# Autodesk Inventor assembly: ASY МОО 001 отстойник осветлитель
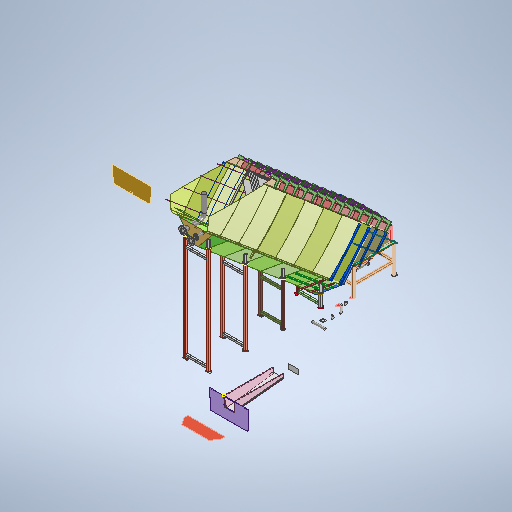
[picture p0: Inventor's stored thumbnail of the model, 512x512]
Saved by Autodesk Inventor 2025 (Build 290162010, 162A)
## iProperties
Created: 2024-04-28
Part Number: ASY МОО 001 отстойник осветлитель
Document SubType Name: Weldment
Designer: admin
Weld Material: Welded Aluminum-6061
Mass: 3.05393e+07 g
Surface Area: 3.06781e+06 cm^2
Volume: 2.84022e+07 cm^3
Density: 1.07525 g/cm^3
Author: admin
## Documents named in this file (70)
- C:\Users\pokla\Documents\Inventor\Отстойник осветлитель\Manturovo_Se-clar-Gleb\ASY MSC 001 отстойник осветлитель.iam
- C:\Users\pokla\Documents\Inventor\Отстойник осветлитель\Manturovo_Se-clar-Gleb\Рама основания\ASY MSC 090 base frame.iam
- C:\Users\pokla\Documents\Inventor\Отстойник осветлитель\Manturovo_Se-clar-Gleb\ASY MSC 080 roсket.iam
- C:\Users\pokla\Documents\Inventor\Отстойник осветлитель\Manturovo_Se-clar-Gleb\ASY MSC 010 cone.iam
- C:\Users\pokla\Documents\Inventor\Отстойник осветлитель\Manturovo_Se-clar-Gleb\ракета\МОО 064 ракета труба.ipt
- C:\Users\pokla\Documents\Inventor\Отстойник осветлитель\Manturovo_Se-clar-Gleb\MSC 000 DIM settler-clarifier.ipt
- C:\Users\pokla\Documents\Inventor\Отстойник осветлитель\Manturovo_Se-clar-Gleb\MSC 031 sheet lowerback.ipt
- C:\Users\pokla\Documents\Inventor\Отстойник осветлитель\Manturovo_Se-clar-Gleb\MSC 021 sheet left board hip.ipt
- C:\Users\pokla\Documents\Inventor\Отстойник осветлитель\Manturovo_Se-clar-Gleb\MSC 022 sheet right board hip.ipt
- C:\Users\pokla\Documents\Inventor\Отстойник осветлитель\Manturovo_Se-clar-Gleb\конус\MSC 071 ridge 1.ipt
- C:\Users\pokla\Documents\Inventor\Отстойник осветлитель\Manturovo_Se-clar-Gleb\конус\MSC 073 ridge 3.ipt
- C:\Users\pokla\Documents\Inventor\Отстойник осветлитель\Manturovo_Se-clar-Gleb\конус\MSC 074 face 1.ipt
- C:\Users\pokla\Documents\Inventor\Отстойник осветлитель\Manturovo_Se-clar-Gleb\Content Center Files\en-US\ISO 5251 B 3D\ISO 5251 Bends 3D without straight ends(90 deg) DN150 11 11.ipt
- C:\Users\pokla\Documents\Inventor\Отстойник осветлитель\Manturovo_Se-clar-Gleb\Content Center Files\en-US\DIN EN 1092-1 01 - PN 25\DIN EN 1092-1 Plate Flange for Welding Type 01 - PN 25 150 x 168.3.ipt
- C:\Users\pokla\Documents\Inventor\Отстойник осветлитель\Manturovo_Se-clar-Gleb\МОО 061 труба верх 1.ipt
- C:\Users\pokla\Documents\Inventor\Отстойник осветлитель\Manturovo_Se-clar-Gleb\МОО 062 труба верх 2.ipt
- C:\Users\pokla\Documents\Inventor\Отстойник осветлитель\Manturovo_Se-clar-Gleb\МОО 063 труба верх 3.ipt
- C:\Users\pokla\Documents\Inventor\Отстойник осветлитель\Manturovo_Se-clar-Gleb\Part1.ipt
- C:\Users\pokla\Documents\Inventor\Отстойник осветлитель\Manturovo_Se-clar-Gleb\MSC 0101 sheet gills.ipt
- C:\Users\pokla\Documents\Inventor\Отстойник осветлитель\Manturovo_Se-clar-Gleb\MSC 068 stringer lowerback.ipt
- C:\Users\pokla\Documents\Inventor\Отстойник осветлитель\Manturovo_Se-clar-Gleb\конус\MSC 072 ridge 2.ipt
- C:\Users\pokla\Documents\Inventor\Отстойник осветлитель\Manturovo_Se-clar-Gleb\MSC 075 face 2.ipt
- C:\Users\pokla\Documents\Inventor\Отстойник осветлитель\Manturovo_Se-clar-Gleb\MSC 076 face 3.ipt
- C:\Users\pokla\Documents\Inventor\Отстойник осветлитель\Manturovo_Se-clar-Gleb\MSC 077 face 4.ipt
- C:\Users\pokla\Documents\Inventor\Отстойник осветлитель\Manturovo_Se-clar-Gleb\MSC 110 revision hatch 1.ipt
- C:\Users\pokla\Documents\Inventor\Отстойник осветлитель\Manturovo_Se-clar-Gleb\MSC 035 ring.ipt
- C:\Users\pokla\Documents\Inventor\Отстойник осветлитель\Manturovo_Se-clar-Gleb\MSC 074 ridge 4.ipt
- C:\Users\pokla\Documents\Inventor\Отстойник осветлитель\Manturovo_Se-clar-Gleb\MSC 075 ridge 5.ipt
- C:\Users\pokla\Documents\Inventor\Отстойник осветлитель\Manturovo_Se-clar-Gleb\MSC 081 pillar 1.ipt
- C:\Users\pokla\Documents\Inventor\Отстойник осветлитель\Manturovo_Se-clar-Gleb\MSC 036 flange 500.ipt
- C:\Users\pokla\Documents\Inventor\Отстойник осветлитель\Manturovo_Se-clar-Gleb\MSC 037 flange cover 500.ipt
- C:\Users\pokla\Documents\Inventor\Отстойник осветлитель\Manturovo_Se-clar-Gleb\MSC 038 flange cover ring 500.ipt
- C:\Users\pokla\Documents\Inventor\Отстойник осветлитель\Manturovo_Se-clar-Gleb\MSC 039 flange cover plate 500.ipt
- C:\Users\pokla\Documents\Inventor\Отстойник осветлитель\Manturovo_Se-clar-Gleb\Рама основания\ASY MSC 120  base frame.iam
- C:\Users\pokla\Documents\Inventor\Отстойник осветлитель\Manturovo_Se-clar-Gleb\Рама основания\ASY MSC 121  base frame.iam
- C:\Users\pokla\Documents\Inventor\Отстойник осветлитель\Manturovo_Se-clar-Gleb\Чертеж для парам. рамы.ipt
- C:\Users\pokla\Documents\Inventor\Отстойник осветлитель\Manturovo_Se-clar-Gleb\ASY MSC 120.1  base frame.iam
- C:\Users\pokla\Documents\Inventor\Отстойник осветлитель\Manturovo_Se-clar-Gleb\ASY MSC 122  base frame.iam
- C:\Users\pokla\Documents\Inventor\Отстойник осветлитель\Manturovo_Se-clar-Gleb\ASY MSC 201 BACK.iam
- C:\Users\pokla\Documents\Inventor\Отстойник осветлитель\Manturovo_Se-clar-Gleb\ASY MSC 202 LEFT BOARD.iam
- C:\Users\pokla\Documents\Inventor\Отстойник осветлитель\Manturovo_Se-clar-Gleb\ASY MSC 203 RIGHT BOARD.iam
- C:\Users\pokla\Documents\Inventor\Отстойник осветлитель\Manturovo_Se-clar-Gleb\ASY MSC 204 BELLY.iam
- C:\Users\pokla\Documents\Inventor\Отстойник осветлитель\Manturovo_Se-clar-Gleb\MSC 063 stringer board #.ipt
- C:\Users\pokla\Documents\Inventor\Отстойник осветлитель\Manturovo_Se-clar-Gleb\MSC 064 stringer board ##.ipt
- C:\Users\pokla\Documents\Inventor\Отстойник осветлитель\Manturovo_Se-clar-Gleb\MSC 055 rib hip 2.ipt
- C:\Users\pokla\Documents\Inventor\Отстойник осветлитель\Manturovo_Se-clar-Gleb\MSC 054 rib hip 1.ipt
- C:\Users\pokla\Documents\Inventor\Отстойник осветлитель\Manturovo_Se-clar-Gleb\MSC 0102 sheet gills.ipt
- C:\Users\pokla\Documents\Inventor\Отстойник осветлитель\Manturovo_Se-clar-Gleb\MSC 078 creen pillar.iam
- C:\Users\pokla\Documents\Inventor\Отстойник осветлитель\Manturovo_Se-clar-Gleb\MSC 0202 sheet gills.ipt
- C:\Users\pokla\Documents\Inventor\Отстойник осветлитель\Manturovo_Se-clar-Gleb\MSC 0103 sheet gills.ipt
- C:\Users\pokla\Documents\Inventor\Отстойник осветлитель\Manturovo_Se-clar-Gleb\MSC 0203 sheet gills.ipt
- C:\Users\pokla\Documents\Inventor\Отстойник осветлитель\Manturovo_Se-clar-Gleb\MSC 0104 sheet gills.ipt
- C:\Users\pokla\Documents\Inventor\Отстойник осветлитель\Manturovo_Se-clar-Gleb\MSC 0204 sheet gills.ipt
- C:\Users\pokla\Documents\Inventor\Отстойник осветлитель\Manturovo_Se-clar-Gleb\MSC 0105 sheet gills.ipt
- C:\Users\pokla\Documents\Inventor\Отстойник осветлитель\Manturovo_Se-clar-Gleb\MSC 0205 sheet gills.ipt
- C:\Users\pokla\Documents\Inventor\Отстойник осветлитель\Manturovo_Se-clar-Gleb\MSC 0106 sheet gills.ipt
- C:\Users\pokla\Documents\Inventor\Отстойник осветлитель\Manturovo_Se-clar-Gleb\MSC 0206 sheet gills.ipt
- C:\Users\pokla\Documents\Inventor\Отстойник осветлитель\Manturovo_Se-clar-Gleb\MSC 0107 sheet gills.ipt
- C:\Users\pokla\Documents\Inventor\Отстойник осветлитель\Manturovo_Se-clar-Gleb\MSC 0207 sheet gills.ipt
- C:\Users\pokla\Documents\Inventor\Отстойник осветлитель\Manturovo_Se-clar-Gleb\MSC 079 creen pillar.ipt
- C:\Users\pokla\Documents\Inventor\Отстойник осветлитель\Manturovo_Se-clar-Gleb\ASY MSC 120 support.iam
- C:\Users\pokla\Documents\Inventor\Отстойник осветлитель\Manturovo_Se-clar-Gleb\ракета\МОО 065 ракета труба 5.ipt
- C:\Users\pokla\Documents\Inventor\Отстойник осветлитель\Manturovo_Se-clar-Gleb\ракета\МОО 066 ракета труба 6.ipt
- C:\Users\pokla\Documents\Inventor\Отстойник осветлитель\Manturovo_Se-clar-Gleb\ракета\МОО 067 ракета труба 7.ipt
- C:\Users\pokla\Documents\Inventor\Отстойник осветлитель\Manturovo_Se-clar-Gleb\ракета\МОО 068 ракета труба 8.ipt
- C:\Users\pokla\Documents\Inventor\Отстойник осветлитель\Manturovo_Se-clar-Gleb\ракета\МОО 069 ракета труба 9.ipt
- C:\Users\pokla\Documents\Inventor\Отстойник осветлитель\Manturovo_Se-clar-Gleb\Content Center Files\en-US\DIN EN 1092-1 01 - PN 25\DIN EN 1092-1 Plate Flange for Welding Type 01 - PN 25 80 x 88.9.ipt
- C:\Users\pokla\Documents\Inventor\Отстойник осветлитель\Manturovo_Se-clar-Gleb\MSC 0391 flange.ipt
- C:\Users\pokla\Documents\Inventor\Отстойник осветлитель\Manturovo_Se-clar-Gleb\MSC 0392 flange 2.ipt
- C:\Users\pokla\Documents\Inventor\Отстойник осветлитель\Manturovo_Se-clar-Gleb\ASY MSC 0130 cone exit back.iam
## Components (95 placed, 72 different names)
1. MSC 000 DIM settler-clarifier.ipt:1
2. MSC 001 DIM frame.ipt:1 — Flush:94, Mate:95, Mate:97, Mate:99, Mate:100
3. ASY MSC 120 support:1 [sub-assembly] — Mate:125, Cylindrical:6
4. ASY MSC 120 support:2 [sub-assembly] — Mate:129, Cylindrical:7
5. ASY MSC 120 support:3 [sub-assembly] — Mate:130, Cylindrical:8
6. ASY MSC 120 support:4 [sub-assembly] — Mate:131, Cylindrical:9
7. MSC 078 creen pillar:1 [sub-assembly]
8. ASY MSC 204 BELLY:1 [sub-assembly] — Mate:125, Mate:129, Mate:130, Mate:131, Mate:132, Mate:133, Mate:135, Flush:102, Mate:137, Mate:139
9. ASY MSC 203 RIGHT BOARD:1 [sub-assembly] — Mate:137, Mate:138
10. ASY MSC 202 LEFT BOARD:1 [sub-assembly]
11. ASY MSC 201 BACK:1 [sub-assembly] — Mate:134, Mate:138, Mate:139
12. ASY MSC 122  base frame:2 [sub-assembly] — Flush:97, Mate:102, Cylindrical:9
13. ASY MSC 120.1  base frame:2 [sub-assembly] — Flush:96, Mate:100, Mate:101, Cylindrical:7
14. ASY MSC 121  base frame:1 [sub-assembly] — Mate:98, Flush:95, Mate:99, Cylindrical:8
15. ASY MSC 120  base frame:1 [sub-assembly] — Flush:93, Mate:97, Cylindrical:6, Cylindrical:10
16. ASY MSC 080 roсket.iam:1 [sub-assembly] — Flush:23
17. ASY MSC 010 cone.iam:1 [sub-assembly] — Flush:22, Mate:16, Flush:28, Mate:65, Mate:78, Tangent:11, Flush:79, Mate:83, Flush:100
18. ASY MSC 090 base frame.iam:1 [sub-assembly] — Flush:19, Flush:21, Flush:82, Flush:100
19. МОО 064 ракета труба.ipt:1 — Rigid:212
20. MSC 031 sheet lowerback.ipt:1 — Mate:15, Mate:16, Tangent:10, Tangent:11, Tangent:12, Cylindrical:2, Rigid:185, Mate:134
21. MSC 021 sheet left board hip.ipt:1 — Flush:41, Mate:78
22. MSC 022 sheet right board hip.ipt:1 — Mate:30
23. MSC 071 ridge 1.ipt:1 — Mate:50, Rigid:211
24. MSC 073 ridge 3.ipt:1 — Rotational:6, Rigid:210, Rigid:211
25. MSC 072 ridge 2.ipt:1 — Rotational:6
26. MSC 077 face 4.ipt:1
27. MSC 074 ridge 4:1 — Rigid:210
28. MSC 075 ridge 5:1
29. MSC 074 face 1.ipt:1 — Rigid:156, Rigid:157, Flush:62, Rigid:159, Mate:132, Mate:133
30. МОО 061 труба верх 1.ipt:1 — Rigid:59, Rigid:159, Rotational:7
31. ISO 5251 Bends 3D without straight ends(90 deg) DN150 11 11.ipt:1 — Rigid:59, Rotational:2
32. МОО 062 труба верх 2.ipt:1 — Rigid:132, Rigid:156
33. DIN EN 1092-1 Plate Flange for Welding Type 01 - PN 25 150 x 168.3.ipt:2 — Rigid:132
34. МОО 063 труба верх 3.ipt:1 — Rigid:157, Rotational:5
35. Part1.ipt:1
36. MSC 068 stringer lowerback.ipt:1 — Mate:65, Tangent:10
37. МОО 061 труба верх 1.ipt:2 — Rotational:2
38. MSC 075 face 2.ipt:1 — Flush:61
39. MSC 076 face 3.ipt:1 — Flush:76
40. MSC 110 revision hatch 1:1 — Flush:82
41. MSC 068 stringer lowerback:2 — Mate:83, Tangent:12
42. MSC 035 ring:1 — Cylindrical:2, Rigid:185, Rigid:186
43. MSC 081 pillar 1:1
44. MSC 036 flange 500:1 — Rigid:175
45. MSC 036 flange 500:2 — Rigid:175, Rigid:176, Rigid:186
46. MSC 036 flange 500:3 — Rigid:176, Rigid:177, Mate:87
47. MSC 036 flange 500:4 — Rigid:177, Rotational:4
48. MSC 037 flange cover 500:1 — Rotational:4, Mate:87, Rigid:178, Mate:108
49. MSC 038 flange cover ring 500:1 — Rigid:178, Mate:109, Tangent:15
50. MSC 055 rib hip 2:2
51. MSC 063 stringer board #.ipt:2
52. MSC 064 stringer board ##.ipt:2
53. MSC 054 rib board hip 1:2
54. MSC 063 stringer board #.ipt:1
55. MSC 054 rib board hip 1:1
56. MSC 055 rib hip 2:1
57. MSC 064 stringer board ##.ipt:1
58. MSC 0102 sheet gills:1 — Rigid:197, Mate:124
59. MSC 0101 sheet gills.ipt:1
60. MSC 0202 sheet gills:1 — Rigid:197
61. MSC 0103 sheet gills:1 — Rigid:199, Mate:123, Mate:124
62. MSC 0203 sheet gills:1 — Rigid:199
63. MSC 0104 sheet gills:1 — Rigid:201, Mate:122, Mate:123
64. MSC 0204 sheet gills:1 — Rigid:201
65. MSC 0105 sheet gills:1 — Rigid:203, Mate:121, Mate:122
66. MSC 0205 sheet gills:1 — Rigid:203
67. MSC 0106 sheet gills:1 — Rigid:205, Mate:120, Mate:121
68. MSC 0206 sheet gills:1 — Rigid:205
69. MSC 0107 sheet gills:1 — Rigid:206, Mate:120
70. MSC 0207 sheet gills:1 — Rigid:206
71. MSC 079 creen pillar:2
72. МОО 064 ракета труба:2
73. МОО 065 ракета труба 5:1 — Rigid:209, Rotational:8
74. МОО 066 ракета труба 6:1
75. МОО 067 ракета труба 7:1 — Rigid:209
76. МОО 068 ракета труба 8:1
77. МОО 069 ракета труба 9:1
78. ASY MSC 120 support:5 [sub-assembly] — Cylindrical:10, Mate:135
79. DIN EN 1092-1 Plate Flange for Welding Type 01 - PN 25 80 x 88.9:1 — Rotational:5
80. DIN EN 1092-1 Plate Flange for Welding Type 01 - PN 25 150 x 168.3:3 — Rotational:7
81. MSC 0391 flange:1 — Rotational:8
82. MSC 0392 flange 2:1 — Rigid:212
83. ASY MSC 0130 cone exit back:1 [sub-assembly]
84. MSC 039 flange cover plate 500:1 — Mate:108, Mate:109, Tangent:15
85. MSC 039 flange cover plate 500:2
86. MSC 039 flange cover plate 500:3
87. MSC 039 flange cover plate 500:4
88. MSC 039 flange cover plate 500:5
89. MSC 039 flange cover plate 500:6
90. MSC 039 flange cover plate 500:7
91. MSC 039 flange cover plate 500:8
92. MSC 039 flange cover plate 500:9
93. MSC 039 flange cover plate 500:10
94. MSC 039 flange cover plate 500:11
95. MSC 039 flange cover plate 500:12
## Component patterns: (12 elements, first: MSC 039 flange cover plate 500:1)
## Relationships (102: Mate 38, WeldJoint 27, Flush 20, RevoluteJoint 6, CylindricalJoint 6, Tangent 4, Angle 1)
- [Flush]: ASY MSC 201 BACK:1
- Flush:19: ASY MSC 090 base frame.iam:1
- Flush:21: ASY MSC 090 base frame.iam:1
- Flush:22: ASY MSC 010 cone.iam:1
- Flush:23: ASY MSC 080 roсket.iam:1
- Mate:15: MSC 031 sheet lowerback.ipt:1
- Mate:16: ASY MSC 010 cone.iam:1 ↔ MSC 031 sheet lowerback.ipt:1
- Flush:28: ASY MSC 010 cone.iam:1
- [Flush]: ASY MSC 202 LEFT BOARD:1
- Flush:41: MSC 021 sheet left board hip.ipt:1
- Mate:30: MSC 022 sheet right board hip.ipt:1
- Mate:50 (200 mm): MSC 071 ridge 1.ipt:1
- Rigid:59 [WeldJoint]: МОО 061 труба верх 1.ipt:1 ↔ ISO 5251 Bends 3D without straight ends(90 deg) DN150 11 11.ipt:1
- Rigid:132 [WeldJoint]: МОО 062 труба верх 2.ipt:1 ↔ DIN EN 1092-1 Plate Flange for Welding Type 01 - PN 25 150 x 168.3.ipt:2
- Mate:65: ASY MSC 010 cone.iam:1 ↔ MSC 068 stringer lowerback.ipt:1
- [Mate]: ASY MSC 201 BACK:1 ↔ MSC 068 stringer lowerback.ipt:1
- Tangent:10: MSC 031 sheet lowerback.ipt:1 ↔ MSC 068 stringer lowerback.ipt:1
- Rotational:2 [RevoluteJoint]: ISO 5251 Bends 3D without straight ends(90 deg) DN150 11 11.ipt:1 ↔ МОО 061 труба верх 1.ipt:2
- Flush:61: MSC 075 face 2.ipt:1
- Rigid:156 [WeldJoint]: MSC 074 face 1.ipt:1 ↔ МОО 062 труба верх 2.ipt:1
- Rigid:157 [WeldJoint]: MSC 074 face 1.ipt:1 ↔ МОО 063 труба верх 3.ipt:1
- Flush:62: MSC 074 face 1.ipt:1
- Rigid:159 [WeldJoint] (-200 mm): MSC 074 face 1.ipt:1 ↔ МОО 061 труба верх 1.ipt:1
- Flush:76: MSC 076 face 3.ipt:1
- Mate:78: ASY MSC 010 cone.iam:1 ↔ MSC 021 sheet left board hip.ipt:1
- Tangent:11 (22 mm): ASY MSC 010 cone.iam:1 ↔ MSC 031 sheet lowerback.ipt:1
- Flush:79: ASY MSC 010 cone.iam:1
- Flush:82: ASY MSC 090 base frame.iam:1 ↔ MSC 110 revision hatch 1:1
- Mate:83: ASY MSC 010 cone.iam:1 ↔ MSC 068 stringer lowerback:2
- [Mate]: ASY MSC 201 BACK:1 ↔ MSC 068 stringer lowerback:2
- Tangent:12: MSC 031 sheet lowerback.ipt:1 ↔ MSC 068 stringer lowerback:2
- Rigid:175 [WeldJoint]: MSC 036 flange 500:1 ↔ MSC 036 flange 500:2
- Rigid:176 [WeldJoint]: MSC 036 flange 500:2 ↔ MSC 036 flange 500:3
- Rigid:177 [WeldJoint]: MSC 036 flange 500:3 ↔ MSC 036 flange 500:4
- Cylindrical:2: MSC 031 sheet lowerback.ipt:1 ↔ MSC 035 ring:1
- Rotational:4 [RevoluteJoint]: MSC 036 flange 500:4 ↔ MSC 037 flange cover 500:1
- Mate:87: MSC 036 flange 500:3 ↔ MSC 037 flange cover 500:1
- Rigid:178 [WeldJoint]: MSC 037 flange cover 500:1 ↔ MSC 038 flange cover ring 500:1
- Flush:93 (-3 mm): ASY MSC 120  base frame:1
- [Mate]: ASY MSC 120  base frame:1
- Flush:94: MSC 001 DIM frame.ipt:1
- Mate:95: MSC 001 DIM frame.ipt:1
- Mate:97: MSC 001 DIM frame.ipt:1 ↔ ASY MSC 120  base frame:1
- Mate:98: ASY MSC 121  base frame:1
- Flush:95 (-3 mm): ASY MSC 121  base frame:1
- Mate:99: MSC 001 DIM frame.ipt:1 ↔ ASY MSC 121  base frame:1
- Flush:96 (-3 mm): ASY MSC 120.1  base frame:2
- Mate:100: MSC 001 DIM frame.ipt:1 ↔ ASY MSC 120.1  base frame:2
- Mate:101: ASY MSC 120.1  base frame:2
- Flush:97 (-3 mm): ASY MSC 122  base frame:2
- Mate:102: ASY MSC 122  base frame:2
- Rigid:185 [WeldJoint] (20 mm): MSC 031 sheet lowerback.ipt:1 ↔ MSC 035 ring:1
- Mate:108: MSC 037 flange cover 500:1 ↔ MSC 039 flange cover plate 500:1
- Mate:109: MSC 038 flange cover ring 500:1 ↔ MSC 039 flange cover plate 500:1
- Tangent:15: MSC 038 flange cover ring 500:1 ↔ MSC 039 flange cover plate 500:1
- Rigid:186 [WeldJoint]: MSC 035 ring:1 ↔ MSC 036 flange 500:2
- [WeldJoint] (500 mm): MSC 054 rib board hip 1:1 ↔ MSC 055 rib hip 2:1
- [WeldJoint] (2 mm): ASY MSC 202 LEFT BOARD:1 ↔ MSC 064 stringer board ##.ipt:2
- [WeldJoint] (500 mm): ASY MSC 202 LEFT BOARD:1 ↔ MSC 055 rib hip 2:2
- [WeldJoint] (500 mm): MSC 055 rib hip 2:2 ↔ MSC 054 rib board hip 1:2
- Rigid:197 [WeldJoint]: MSC 0102 sheet gills:1 ↔ MSC 0202 sheet gills:1
- Rigid:199 [WeldJoint]: MSC 0103 sheet gills:1 ↔ MSC 0203 sheet gills:1
- Rigid:201 [WeldJoint]: MSC 0104 sheet gills:1 ↔ MSC 0204 sheet gills:1
- Rigid:203 [WeldJoint]: MSC 0105 sheet gills:1 ↔ MSC 0205 sheet gills:1
- Rigid:205 [WeldJoint]: MSC 0106 sheet gills:1 ↔ MSC 0206 sheet gills:1
- Rigid:206 [WeldJoint]: MSC 0107 sheet gills:1 ↔ MSC 0207 sheet gills:1
- Mate:120 (50 mm): MSC 0106 sheet gills:1 ↔ MSC 0107 sheet gills:1
- Mate:121 (50 mm): MSC 0105 sheet gills:1 ↔ MSC 0106 sheet gills:1
- Mate:122 (50 mm): MSC 0104 sheet gills:1 ↔ MSC 0105 sheet gills:1
- Mate:123 (50 mm): MSC 0103 sheet gills:1 ↔ MSC 0104 sheet gills:1
- Mate:124 (50 mm): MSC 0102 sheet gills:1 ↔ MSC 0103 sheet gills:1
- Mate:125: ASY MSC 120 support:1 ↔ ASY MSC 204 BELLY:1
- [Mate]: ASY MSC 204 BELLY:1 ↔ ASY MSC 0130 cone exit back:1
- [Angle] (0 deg): ASY MSC 204 BELLY:1 ↔ ASY MSC 0130 cone exit back:1
- Flush:100: ASY MSC 010 cone.iam:1 ↔ ASY MSC 090 base frame.iam:1
- Cylindrical:6: ASY MSC 120 support:1 ↔ ASY MSC 120  base frame:1
- Mate:129: ASY MSC 120 support:2 ↔ ASY MSC 204 BELLY:1
- Mate:130: ASY MSC 120 support:3 ↔ ASY MSC 204 BELLY:1
- Mate:131: ASY MSC 120 support:4 ↔ ASY MSC 204 BELLY:1
- Cylindrical:7: ASY MSC 120 support:2 ↔ ASY MSC 120.1  base frame:2
- Cylindrical:8: ASY MSC 120 support:3 ↔ ASY MSC 121  base frame:1
- Cylindrical:9: ASY MSC 120 support:4 ↔ ASY MSC 122  base frame:2
- Mate:132: ASY MSC 204 BELLY:1 ↔ MSC 074 face 1.ipt:1
- Mate:133: ASY MSC 204 BELLY:1 ↔ MSC 074 face 1.ipt:1
- Mate:134: ASY MSC 201 BACK:1 ↔ MSC 031 sheet lowerback.ipt:1
- [WeldJoint]: ASY MSC 010 cone.iam:1 ↔ ASY MSC 0130 cone exit back:1
- [WeldJoint]: МОО 067 ракета труба 7:1 ↔ ASY MSC 0130 cone exit back:1
- Rigid:209 [WeldJoint]: МОО 065 ракета труба 5:1 ↔ МОО 067 ракета труба 7:1
- Cylindrical:10: ASY MSC 120  base frame:1 ↔ ASY MSC 120 support:5
- Mate:135: ASY MSC 204 BELLY:1 ↔ ASY MSC 120 support:5
- Flush:102: ASY MSC 204 BELLY:1
- [Mate]: ASY MSC 203 RIGHT BOARD:1 ↔ ASY MSC 0130 cone exit back:1
- Mate:137: ASY MSC 204 BELLY:1 ↔ ASY MSC 203 RIGHT BOARD:1
- Mate:138: ASY MSC 203 RIGHT BOARD:1 ↔ ASY MSC 201 BACK:1
- Mate:139 (-2857 mm): ASY MSC 204 BELLY:1 ↔ ASY MSC 201 BACK:1
- Rotational:5 [RevoluteJoint]: МОО 063 труба верх 3.ipt:1 ↔ DIN EN 1092-1 Plate Flange for Welding Type 01 - PN 25 80 x 88.9:1
- Rotational:6 [RevoluteJoint]: MSC 073 ridge 3.ipt:1 ↔ MSC 072 ridge 2.ipt:1
- Rigid:210 [WeldJoint]: MSC 073 ridge 3.ipt:1 ↔ MSC 074 ridge 4:1
- Rigid:211 [WeldJoint]: MSC 071 ridge 1.ipt:1 ↔ MSC 073 ridge 3.ipt:1
- Rotational:7 [RevoluteJoint]: МОО 061 труба верх 1.ipt:1 ↔ DIN EN 1092-1 Plate Flange for Welding Type 01 - PN 25 150 x 168.3:3
- Rotational:8 [RevoluteJoint] (30 mm): МОО 065 ракета труба 5:1 ↔ MSC 0391 flange:1
- Rigid:212 [WeldJoint] (30 mm): МОО 064 ракета труба.ipt:1 ↔ MSC 0392 flange 2:1
## Named parameters: Бак_нахлест_фланца = 25 mm, Шаг_опор_по_баку = 2000 mm
